# Autodesk Inventor assembly: ASY Обрешетка лицевая стенка
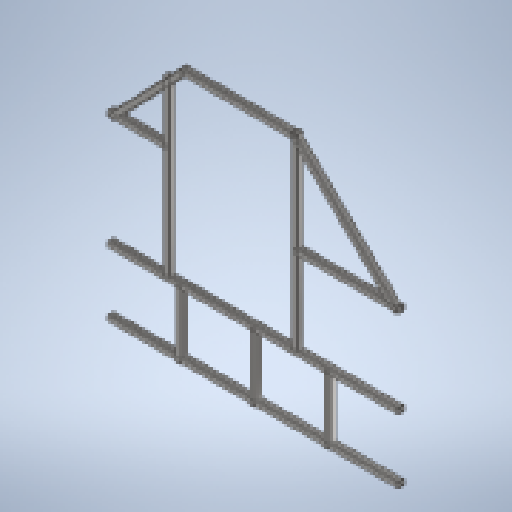
[picture p0: Inventor's stored thumbnail of the model, 512x512]
Saved by Autodesk Inventor 2026.3 (Build 303398000, 398)
## iProperties
_SolveAssemblyDoc: Frame Generator Solve Assembly
_Version: 25.0.0
Created: 2025-08-19
Part Number: ASY Обрешетка лицевая стенка
Document SubType Name: Assembly
Designer: pokla
Author: pokla
## Documents named in this file (3)
- C:\Users\admin\Documents\Inventor\DMF-Disk-Micro-Filter\ASY Обрешетка лицевая стенка.iam
- C:\Users\admin\Documents\Inventor\DMF-Disk-Micro-Filter\Обрешетка_лицевая_стенка_скетч.ipt
- C:\Users\admin\Documents\Inventor\DMF-Disk-Micro-Filter\Обрешетка лицевая стенка\Frame\Frame 1755631368535.iam
## Components (2 placed, 2 different names)
1. Обрешетка_лицевая_стенка_скетч.ipt:1 — Mate:1
2. Frame 1755631368535.iam:1 [sub-assembly] — Mate:1
## Relationships (1: Mate 1)
- Mate:1: Обрешетка_лицевая_стенка_скетч.ipt:1 ↔ Frame 1755631368535.iam:1
